# Autodesk Inventor assembly: legg_assembly
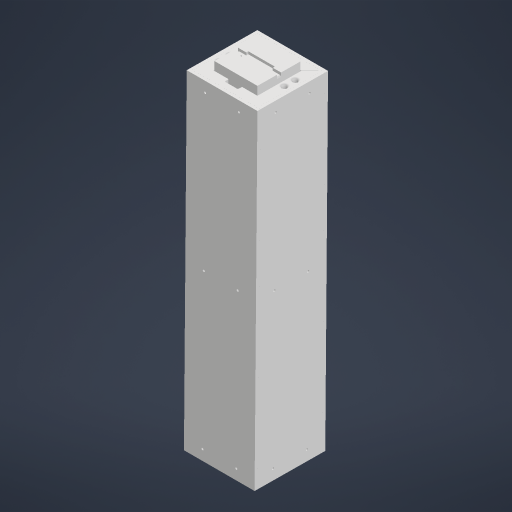
[picture p0: Inventor's stored thumbnail of the model, 512x512]
Saved by Autodesk Inventor 2024 (Build 280153000, 153)
## iProperties
Created: 2023-05-23
Part Number: legg_assembly
Document SubType Name: Assembly
Designer: aasmu
Author: aasmu
## Documents named in this file (5)
- C:\Users\aasmu\Documents\standing_desk\12_legg_assembly.iam
- C:\Users\aasmu\Documents\standing_desk\01_inner_leg.ipt
- C:\Users\aasmu\Documents\standing_desk\00_inner_leg_top_plate.ipt
- C:\Users\aasmu\Documents\standing_desk\13_centerlegg_assembly.iam
- C:\Users\aasmu\Documents\standing_desk\14_outerlegg_assembly.iam
## Components (4 placed, 4 different names)
1. 01_inner_leg:1 — Rigid:1, Mate:1, Mate:2
2. 00_inner_leg_top_plate:1 — Rigid:1
3. 13_centerlegg_assembly:1 [sub-assembly] — Mate:1, Mate:2, Mate:3, Mate:4
4. 14_outerlegg_assembly:1 [sub-assembly] — Mate:3, Mate:4
## Relationships (5: Mate 4, WeldJoint 1)
- Rigid:1 [WeldJoint]: 01_inner_leg:1 ↔ 00_inner_leg_top_plate:1
- Mate:1: 01_inner_leg:1 ↔ 13_centerlegg_assembly:1
- Mate:2: 01_inner_leg:1 ↔ 13_centerlegg_assembly:1
- Mate:3: 13_centerlegg_assembly:1 ↔ 14_outerlegg_assembly:1
- Mate:4: 13_centerlegg_assembly:1 ↔ 14_outerlegg_assembly:1
